# Autodesk Inventor assembly: Superior do cilindro 3
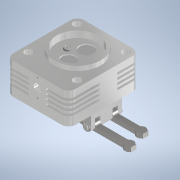
[picture p0: Inventor's stored thumbnail of the model, 180x180]
Saved by Autodesk Inventor 2021 (Build 250183000, 183)
## iProperties
Created: 2021-07-22
Part Number: Superior do cilindro 3
Document SubType Name: Assembly
Designer: Giovanni
Author: Giovanni
## Documents named in this file (12)
- C:\Users\irineu\Documents\Inventor\MotorRadial7\Superior do cilindro 3.iam
- C:\Users\irineu\Documents\Inventor\MotorRadial7\Peça5.3.ipt
- C:\Users\irineu\Documents\Inventor\MotorRadial7\Peça7.ipt
- C:\Users\irineu\Documents\Inventor\MotorRadial7\Peça24.ipt
- C:\Users\irineu\Documents\Inventor\MotorRadial7\Peça16.ipt
- C:\Users\irineu\Documents\Inventor\MotorRadial7\Peça17.ipt
- C:\Users\irineu\Documents\Inventor\MotorRadial7\Peça19.ipt
- C:\Users\irineu\Documents\Inventor\MotorRadial7\Peça8.ipt
- C:\Users\irineu\Documents\Inventor\MotorRadial7\Peça9.ipt
- C:\Users\irineu\Documents\Inventor\Content Center Files\R2021\pt-BR\DIN 912\DIN 912 - M4 x 0,7 x 20 x 18,25.ipt
- C:\Users\irineu\Documents\Inventor\MotorRadial7\Peça18.ipt
- C:\Users\irineu\Documents\Inventor\Content Center Files\R2021\pt-BR\DIN 6799\DIN 6799 - 8 12.ipt
## Components (18 placed, 11 different names)
1. Peça5.3:1 — Alinhado:1, Coincidente:1, Alinhado:2, Inserir:1, Inserir:2, Inserir:3, Ângulo:1, Coincidente:2, Coincidente:3, Coincidente:4, Coincidente:5, Coincidente:10, Coincidente:12, Ângulo:2, Ângulo:3
2. Peça7:1 — Inserir:1, Coincidente:9
3. Peça7:2 — Inserir:2, Coincidente:7
4. Peça24:1 — Inserir:3, Ângulo:1
5. Peça16:1 — Coincidente:6, Coincidente:7, Inserir:8
6. Peça16:2 — Coincidente:8, Coincidente:9, Inserir:9
7. Peça17:1 — Coincidente:2, Coincidente:5, Coincidente:8
8. Peça17:2 — Coincidente:3, Coincidente:4, Coincidente:6
9. Peça19:1 — Coincidente:10, Coincidente:11, Coincidente:12, Coincidente:13, Coincidente:14, Coincidente:15, Coincidente:16, Inserir:4, Inserir:5, Coincidente:17
10. Peça8:1 — Coincidente:13, Coincidente:14, Ângulo:2
11. Peça9:1 — Coincidente:15, Coincidente:16, Ângulo:3
12. DIN 912 - substituído por DIN EN ISO 4762 M4 x 20:1 — Inserir:4
13. DIN 912 - substituído por DIN EN ISO 4762 M4 x 20:2 — Inserir:5
14. Peça18:1 — Coincidente:17, Coincidente:18, Inserir:6, Inserir:7
15. DIN 6799 8:3 — Inserir:7
16. DIN 6799 8:4 — Inserir:6
17. DIN 6799 8:5 — Inserir:9
18. DIN 6799 8:6 — Inserir:8
## Relationships (32: Mate 18, Insert 9, Angle 3, Flush 2)
- Alinhado:1 [Flush]: Peça5.3:1
- Coincidente:1 [Mate]: Peça5.3:1
- Alinhado:2 [Flush]: Peça5.3:1
- Inserir:1: Peça5.3:1 ↔ Peça7:1
- Inserir:2: Peça5.3:1 ↔ Peça7:2
- Inserir:3: Peça5.3:1 ↔ Peça24:1
- Ângulo:1 [Angle] (0 deg): Peça5.3:1 ↔ Peça24:1
- Coincidente:2 [Mate]: Peça5.3:1 ↔ Peça17:1
- Coincidente:3 [Mate]: Peça5.3:1 ↔ Peça17:2
- Coincidente:4 [Mate]: Peça5.3:1 ↔ Peça17:2
- Coincidente:5 [Mate]: Peça5.3:1 ↔ Peça17:1
- Coincidente:6 [Mate]: Peça16:1 ↔ Peça17:2
- Coincidente:7 [Mate]: Peça7:2 ↔ Peça16:1
- Coincidente:8 [Mate]: Peça16:2 ↔ Peça17:1
- Coincidente:9 [Mate]: Peça7:1 ↔ Peça16:2
- Coincidente:10 [Mate]: Peça5.3:1 ↔ Peça19:1
- Coincidente:11 [Mate]: Peça19:1
- Coincidente:12 [Mate]: Peça5.3:1 ↔ Peça19:1
- Coincidente:13 [Mate]: Peça19:1 ↔ Peça8:1
- Coincidente:14 [Mate]: Peça19:1 ↔ Peça8:1
- Ângulo:2 [Angle] (0 deg): Peça5.3:1 ↔ Peça8:1
- Coincidente:15 [Mate]: Peça19:1 ↔ Peça9:1
- Coincidente:16 [Mate]: Peça19:1 ↔ Peça9:1
- Ângulo:3 [Angle] (0 deg): Peça5.3:1 ↔ Peça9:1
- Inserir:4: Peça19:1 ↔ DIN 912 - substituído por DIN EN ISO 4762 M4 x 20:1
- Inserir:5: Peça19:1 ↔ DIN 912 - substituído por DIN EN ISO 4762 M4 x 20:2
- Coincidente:17 [Mate]: Peça19:1 ↔ Peça18:1
- Coincidente:18 [Mate]: Peça18:1
- Inserir:6: Peça18:1 ↔ DIN 6799 8:4
- Inserir:7: Peça18:1 ↔ DIN 6799 8:3
- Inserir:8: Peça16:1 ↔ DIN 6799 8:6
- Inserir:9: Peça16:2 ↔ DIN 6799 8:5
